# Autodesk Inventor assembly: PowerHub
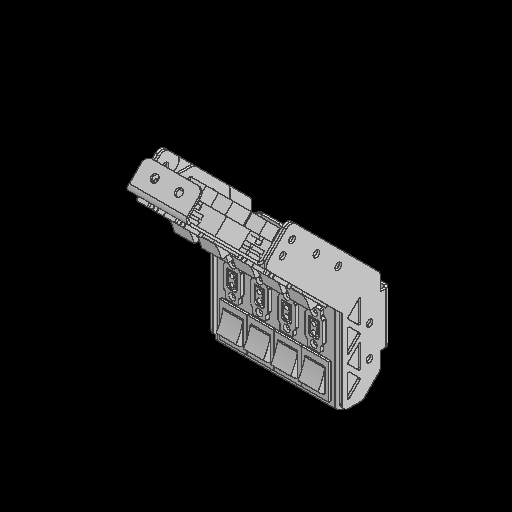
[picture p0: Inventor's stored thumbnail of the model, 512x512]
Saved by Autodesk Inventor 2025.2 (Build 292293000, 293)
## iProperties
Created: 2026-06-06
Part Number: PowerHub
Document SubType Name: Assembly
Designer: valer
Author: valer
## Documents named in this file (7)
- C:\Users\valer\Desktop\str1ker\cad\PowerHub.iam
- C:\Users\valer\Desktop\str1ker\cad\external\XT60E-F.ipt
- C:\Users\valer\Desktop\str1ker\cad\external\IlluminatedSwitch12V10A.ipt
- C:\Users\valer\Desktop\str1ker\cad\PowerHubFrontPanel.ipt
- C:\Users\valer\Desktop\str1ker\cad\PowerHubSide.ipt
- C:\Users\valer\Desktop\str1ker\cad\PowerHubEndPanel.ipt
- C:\Users\valer\Desktop\str1ker\cad\PowerHubSideMirror.ipt
## Components (25 placed, 6 different names)
1. IlluminatedSwitch12V10A:1 — Mate:5, Mate:7, Flush:7, Flush:17, Flush:18, Flush:24, Mate:52, Flush:69, Mate:53
2. XT60E-F:1 — Mate:5, Flush:17, Flush:21, Flush:24, Mate:49
3. IlluminatedSwitch12V10A:2 — Flush:6, Mate:7, Flush:7, Mate:11, Flush:9, Flush:18, Flush:19
4. XT60E-F:2 — Flush:6, Flush:21, Flush:22
5. IlluminatedSwitch12V10A:3 — Mate:11, Flush:9, Flush:11, Mate:15, Flush:19, Flush:20
6. XT60E-F:3 — Flush:22, Flush:23
7. IlluminatedSwitch12V10A:4 — Flush:11, Mate:15, Flush:20
8. XT60E-F:4 — Flush:23
9. IlluminatedSwitch12V10A:5 — Flush:69
10. XT60E-F:5
11. IlluminatedSwitch12V10A:6
12. XT60E-F:6
13. IlluminatedSwitch12V10A:7
14. XT60E-F:7
15. IlluminatedSwitch12V10A:8
16. XT60E-F:8
17. PowerHubFrontPanel:2 — Flush:65, Flush:67, Mate:42, Mate:46, Mate:50, Mate:53
18. IlluminatedSwitch12V10A:10 — Mate:39
19. XT60E-F:10 — Mate:35, Mate:36, Mate:37
20. IlluminatedSwitch12V10A:11
21. XT60E-F:11
22. PowerHubSide:1 — Mate:33, Flush:65, Flush:66, Mate:40, Mate:43, Mate:46
23. PowerHubEndPanel:1 — Mate:33, Mate:35, Mate:36, Mate:37, Mate:39, Flush:66, Flush:68, Mate:44, Mate:45, Mate:51
24. PowerHubSideMirror:1 — Mate:45, Mate:51
25. PowerHubFrontPanel:3 — Mate:42, Mate:43, Flush:68, Mate:44, Mate:49, Mate:52
## Relationships (73: Flush 39, Mate 34)
- Mate:5 (4 mm): IlluminatedSwitch12V10A:1 ↔ XT60E-F:1
- [Mate] (4 mm): IlluminatedSwitch12V10A:2 ↔ XT60E-F:2
- Flush:6: IlluminatedSwitch12V10A:2 ↔ XT60E-F:2
- Mate:7: IlluminatedSwitch12V10A:1 ↔ IlluminatedSwitch12V10A:2
- Flush:7: IlluminatedSwitch12V10A:1 ↔ IlluminatedSwitch12V10A:2
- [Mate] (4 mm): IlluminatedSwitch12V10A:3 ↔ XT60E-F:3
- [Flush]: IlluminatedSwitch12V10A:3 ↔ XT60E-F:3
- Mate:11: IlluminatedSwitch12V10A:2 ↔ IlluminatedSwitch12V10A:3
- Flush:9: IlluminatedSwitch12V10A:2 ↔ IlluminatedSwitch12V10A:3
- [Mate] (4 mm): IlluminatedSwitch12V10A:4 ↔ XT60E-F:4
- [Flush]: IlluminatedSwitch12V10A:4 ↔ XT60E-F:4
- Flush:11: IlluminatedSwitch12V10A:3 ↔ IlluminatedSwitch12V10A:4
- Mate:15: IlluminatedSwitch12V10A:3 ↔ IlluminatedSwitch12V10A:4
- Flush:17: IlluminatedSwitch12V10A:1 ↔ XT60E-F:1
- Flush:18: IlluminatedSwitch12V10A:1 ↔ IlluminatedSwitch12V10A:2
- Flush:19: IlluminatedSwitch12V10A:2 ↔ IlluminatedSwitch12V10A:3
- Flush:20: IlluminatedSwitch12V10A:3 ↔ IlluminatedSwitch12V10A:4
- Flush:21: XT60E-F:1 ↔ XT60E-F:2
- Flush:22: XT60E-F:2 ↔ XT60E-F:3
- Flush:23: XT60E-F:3 ↔ XT60E-F:4
- Flush:24: IlluminatedSwitch12V10A:1 ↔ XT60E-F:1
- [Mate] (4 mm): IlluminatedSwitch12V10A:5 ↔ XT60E-F:5
- [Mate] (4 mm): IlluminatedSwitch12V10A:6 ↔ XT60E-F:6
- [Flush]: IlluminatedSwitch12V10A:6 ↔ XT60E-F:6
- [Mate]: IlluminatedSwitch12V10A:5 ↔ IlluminatedSwitch12V10A:6
- [Flush]: IlluminatedSwitch12V10A:5 ↔ IlluminatedSwitch12V10A:6
- [Mate] (4 mm): IlluminatedSwitch12V10A:7 ↔ XT60E-F:7
- [Flush]: IlluminatedSwitch12V10A:7 ↔ XT60E-F:7
- [Mate]: IlluminatedSwitch12V10A:6 ↔ IlluminatedSwitch12V10A:7
- [Flush]: IlluminatedSwitch12V10A:6 ↔ IlluminatedSwitch12V10A:7
- [Mate] (4 mm): IlluminatedSwitch12V10A:8 ↔ XT60E-F:8
- [Flush]: IlluminatedSwitch12V10A:8 ↔ XT60E-F:8
- [Flush]: IlluminatedSwitch12V10A:7 ↔ IlluminatedSwitch12V10A:8
- [Mate]: IlluminatedSwitch12V10A:7 ↔ IlluminatedSwitch12V10A:8
- [Flush]: IlluminatedSwitch12V10A:5 ↔ XT60E-F:5
- [Flush]: IlluminatedSwitch12V10A:5 ↔ IlluminatedSwitch12V10A:6
- [Flush]: IlluminatedSwitch12V10A:6 ↔ IlluminatedSwitch12V10A:7
- [Flush]: IlluminatedSwitch12V10A:7 ↔ IlluminatedSwitch12V10A:8
- [Flush]: XT60E-F:5 ↔ XT60E-F:6
- [Flush]: XT60E-F:6 ↔ XT60E-F:7
- [Flush]: XT60E-F:7 ↔ XT60E-F:8
- [Flush]: IlluminatedSwitch12V10A:5 ↔ XT60E-F:5
- [Mate]: IlluminatedSwitch12V10A:5 ↔ PowerHubFrontPanel:2
- [Flush] (4 mm): IlluminatedSwitch12V10A:5 ↔ PowerHubFrontPanel:2
- [Mate] (4 mm): IlluminatedSwitch12V10A:10 ↔ XT60E-F:10
- [Flush]: IlluminatedSwitch12V10A:10 ↔ XT60E-F:10
- [Mate] (4 mm): IlluminatedSwitch12V10A:11 ↔ XT60E-F:11
- [Flush]: IlluminatedSwitch12V10A:11 ↔ XT60E-F:11
- [Mate]: IlluminatedSwitch12V10A:10 ↔ IlluminatedSwitch12V10A:11
- [Flush]: IlluminatedSwitch12V10A:10 ↔ IlluminatedSwitch12V10A:11
- [Flush]: IlluminatedSwitch12V10A:10 ↔ IlluminatedSwitch12V10A:11
- [Flush]: XT60E-F:10 ↔ XT60E-F:11
- Mate:33: PowerHubSide:1 ↔ PowerHubEndPanel:1
- Mate:35: XT60E-F:10 ↔ PowerHubEndPanel:1
- Mate:36: XT60E-F:10 ↔ PowerHubEndPanel:1
- Mate:37: XT60E-F:10 ↔ PowerHubEndPanel:1
- Flush:65: PowerHubFrontPanel:2 ↔ PowerHubSide:1
- Mate:39: IlluminatedSwitch12V10A:10 ↔ PowerHubEndPanel:1
- Flush:66: PowerHubSide:1 ↔ PowerHubEndPanel:1
- Mate:40: PowerHubSide:1
- Flush:67: PowerHubFrontPanel:2
- Mate:42: PowerHubFrontPanel:2 ↔ PowerHubFrontPanel:3
- Mate:43: PowerHubSide:1 ↔ PowerHubFrontPanel:3
- Flush:68: PowerHubEndPanel:1 ↔ PowerHubFrontPanel:3
- Mate:44: PowerHubEndPanel:1 ↔ PowerHubFrontPanel:3
- Mate:45: PowerHubEndPanel:1 ↔ PowerHubSideMirror:1
- Mate:46: PowerHubFrontPanel:2 ↔ PowerHubSide:1
- Mate:49: XT60E-F:1 ↔ PowerHubFrontPanel:3
- Mate:50: PowerHubFrontPanel:2
- Mate:51: PowerHubEndPanel:1 ↔ PowerHubSideMirror:1
- Mate:52 (4 mm): IlluminatedSwitch12V10A:1 ↔ PowerHubFrontPanel:3
- Flush:69: IlluminatedSwitch12V10A:1 ↔ IlluminatedSwitch12V10A:5
- Mate:53 (4 mm): IlluminatedSwitch12V10A:1 ↔ PowerHubFrontPanel:2
## Named parameters: d94_d93 = 4 mm, d100_d94_d93 = 4 mm, d101_d95 = 0 mm, d106_d100_d94_d93 = 4 mm, d107_d101_d95 = 0 mm, d183_d173 = 0 mm, d184_d174 = 0 mm, d185_d175 = 0 mm, d186_d176 = 0 mm, d187_d177 = 0 mm, d188_d178 = 0 mm, d189_d179 = 0 mm, d190_d180 = 0 mm, d191_d93 = 4 mm, d192_d94_d93 = 4 mm, d193_d95 = 0 mm, d194_d96 = 0 mm, d195_d97 = 0 mm, d196_d100_d94_d93 = 4 mm, d197_d101_d95 = 0 mm, d198_d102 = 0 mm, d199_d103 = 0 mm, d200_d106_d100_d94_d93 = 4 mm, d201_d107_d101_d95 = 0 mm, d202_d108 = 0 mm, d203_d109 = 0 mm, d204_d123 = 0 mm, d205_d182 = 4 mm, d210_d184_d174 = 0 mm, d213_d187_d177 = 0 mm, d218_d192_d94_d93 = 4 mm, d219_d193_d95 = 0 mm, d222_d196_d100_d94_d93 = 4 mm, d223_d197_d101_d95 = 0 mm, d224_d198_d102 = 0 mm, d225_d199_d103 = 0 mm
